# Autodesk Inventor assembly: GE-12091
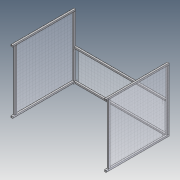
[picture p0: Inventor's stored thumbnail of the model, 180x180]
Saved by Autodesk Inventor 2012 (Build 160160000, 160)
## iProperties
Created: 2011-10-10
Part Number: GE-12091
Document SubType Name: Assembly
Designer: dfoster
Description: Corral Assembly
Title: Corral Assembly
Author: dfoster
## Documents named in this file (7)
- C:\Data Folder\FRC 2012 Field\Components\GE-12091.iam
- C:\Data Folder\FRC 2012 Field\Components\GE-12089.iam
- C:\Data Folder\FRC 2012 Field\Components\GE-12092.iam
- C:\Data Folder\FRC 2012 Field\Components\GE-12093.ipt
- C:\Data Folder\FRC 2012 Field\Components\GE-12094.ipt
- C:\Data Folder\FRC 2012 Field\Components\GE-12090.ipt
- C:\Data Folder\FRC 2012 Field\Components\HW-00005.0005.ipt
## Components (11 placed, 6 different names)
1. GE-12089:1 [sub-assembly] — Flush:1, Flush:2, Mate:1, Mate:3, Flush:8, Flush:9, Mate:5, Mate:7, Mate:9
2. GE-12092:1 [sub-assembly] — Flush:1, Flush:2, Mate:1, Flush:5, Flush:6, Flush:7, Flush:10, Mate:4, Flush:11, Mate:6
3. GE-12093:1 — Flush:5, Flush:6, Flush:7
4. GE-12093:2 — Mate:3, Flush:8, Flush:9
5. GE-12094:1 — Mate:8, Flush:12, Mate:9
6. GE-12090:1 — Flush:11, Mate:6, Mate:7, Insert:2, Insert:4
7. GE-12090:2 — Flush:10, Mate:4, Mate:5, Insert:1, Insert:3, Mate:8, Flush:12
8. HW-00005.0005:1 — Insert:1
9. HW-00005.0005:2 — Insert:2
10. HW-00005.0005:3 — Insert:4
11. HW-00005.0005:4 — Insert:3
## Relationships (22: Flush 10, Mate 8, Insert 4)
- Flush:1: GE-12089:1 ↔ GE-12092:1
- Flush:2: GE-12089:1 ↔ GE-12092:1
- Mate:1 (-1828.8 mm): GE-12089:1 ↔ GE-12092:1
- Flush:5: GE-12092:1 ↔ GE-12093:1
- Flush:6: GE-12092:1 ↔ GE-12093:1
- Flush:7: GE-12092:1 ↔ GE-12093:1
- Mate:3: GE-12089:1 ↔ GE-12093:2
- Flush:8: GE-12089:1 ↔ GE-12093:2
- Flush:9: GE-12089:1 ↔ GE-12093:2
- Flush:10: GE-12092:1 ↔ GE-12090:2
- Mate:4: GE-12092:1 ↔ GE-12090:2
- Mate:5: GE-12089:1 ↔ GE-12090:2
- Flush:11: GE-12092:1 ↔ GE-12090:1
- Mate:6: GE-12092:1 ↔ GE-12090:1
- Mate:7: GE-12089:1 ↔ GE-12090:1
- Insert:1: GE-12090:2 ↔ HW-00005.0005:1
- Insert:2: GE-12090:1 ↔ HW-00005.0005:2
- Insert:3: GE-12090:2 ↔ HW-00005.0005:4
- Insert:4: GE-12090:1 ↔ HW-00005.0005:3
- Mate:8: GE-12094:1 ↔ GE-12090:2
- Flush:12: GE-12094:1 ↔ GE-12090:2
- Mate:9 (57.15 mm): GE-12089:1 ↔ GE-12094:1
